# Autodesk Inventor assembly: Assembly1
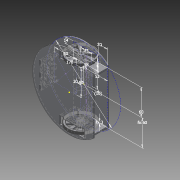
[picture p0: Inventor's stored thumbnail of the model, 180x180]
Saved by Autodesk Inventor 2015 (Build 190159000, 159)
## iProperties
Created: 2014-07-27
Part Number: Assembly1
Document SubType Name: Assembly
Designer: karl
Author: karl
## Documents named in this file (8)
- C:\Users\karl\Documents\GitHub\SUMOChassis\Body\2nd vier\Assembly1.iam
- C:\Users\karl\Documents\GitHub\SUMOChassis\Body\Base Plate.ipt
- C:\Users\karl\Documents\GitHub\SUMOChassis\Body\Motor mount plate.ipt
- C:\Users\karl\Documents\GitHub\SUMOChassis\Body\Motor Side support.ipt
- C:\Users\karl\Documents\GitHub\SUMOChassis\Body\Wheel.ipt
- C:\Users\karl\Documents\GitHub\SUMOChassis\Body\Back Plate.ipt
- C:\Users\karl\Documents\GitHub\SUMOChassis\Body\Motor.ipt
- C:\Users\karl\Documents\GitHub\SUMOChassis\Body\2nd vier\Mid Plate.ipt
## Components (11 placed, 7 different names)
1. Base Plate:1 — Mate:1, Mate:2, Flush:1, Mate:4, Mate:5, Flush:3, Mate:6, Mate:7, Mate:13, Mate:14, Mate:20, Flush:6
2. Motor mount plate:1 — Mate:1, Mate:2, Flush:1, Mate:3, Flush:2, Mate:9, Mate:10, Mate:19
3. Motor Side support:1 — Mate:3, Mate:4, Flush:2
4. Motor Side support:2 — Mate:5, Flush:3, Flush:4, Mate:8
5. Motor mount plate:2 — Mate:6, Mate:7, Flush:4, Mate:8, Mate:11, Mate:12, Flush:5, Mate:15, Mate:16, Mate:17
6. Wheel:1 — Mate:9, Mate:10
7. Wheel:2 — Mate:11, Mate:12
8. Back Plate:1 — Mate:13, Flush:5, Mate:14, Mate:21
9. Motor:1 — Mate:15, Mate:16, Mate:17, Mate:18
10. Motor:2 — Mate:18, Mate:19
11. Mid Plate:1 — Mate:20, Mate:21, Flush:6
## Relationships (27: Mate 21, Flush 6)
- Mate:1: Base Plate:1 ↔ Motor mount plate:1
- Mate:2: Base Plate:1 ↔ Motor mount plate:1
- Flush:1: Base Plate:1 ↔ Motor mount plate:1
- Mate:3: Motor mount plate:1 ↔ Motor Side support:1
- Mate:4: Base Plate:1 ↔ Motor Side support:1
- Flush:2: Motor mount plate:1 ↔ Motor Side support:1
- Mate:5: Base Plate:1 ↔ Motor Side support:2
- Flush:3: Base Plate:1 ↔ Motor Side support:2
- Mate:6: Base Plate:1 ↔ Motor mount plate:2
- Mate:7: Base Plate:1 ↔ Motor mount plate:2
- Flush:4: Motor Side support:2 ↔ Motor mount plate:2
- Mate:8: Motor Side support:2 ↔ Motor mount plate:2
- Mate:9: Motor mount plate:1 ↔ Wheel:1
- Mate:10 (2 mm): Motor mount plate:1 ↔ Wheel:1
- Mate:11 (2 mm): Motor mount plate:2 ↔ Wheel:2
- Mate:12: Motor mount plate:2 ↔ Wheel:2
- Mate:13: Base Plate:1 ↔ Back Plate:1
- Flush:5: Motor mount plate:2 ↔ Back Plate:1
- Mate:14: Base Plate:1 ↔ Back Plate:1
- Mate:15: Motor mount plate:2 ↔ Motor:1
- Mate:16: Motor mount plate:2 ↔ Motor:1
- Mate:17: Motor mount plate:2 ↔ Motor:1
- Mate:18: Motor:1 ↔ Motor:2
- Mate:19: Motor mount plate:1 ↔ Motor:2
- Mate:20: Base Plate:1 ↔ Mid Plate:1
- Mate:21: Back Plate:1 ↔ Mid Plate:1
- Flush:6: Base Plate:1 ↔ Mid Plate:1
